# Autodesk Inventor assembly: A Drive
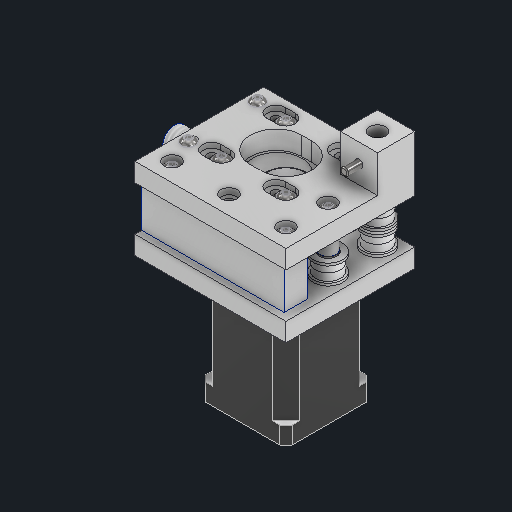
[picture p0: Inventor's stored thumbnail of the model, 512x512]
Saved by Autodesk Inventor 2025.1 (Build 291241020, 241B)
## iProperties
Created: 2025-05-09
Part Number: A Drive
Document SubType Name: Assembly
Designer: AdminForWorker
Title: A Drive
Author: AdminForWorker
## Documents named in this file (9)
- C:\Users\Joshua Eah\Documents\Voron 0.2\CAD\Master Assembly\Motion\AB Drives\A Drive.iam
- C:\Users\Joshua Eah\Documents\Voron 0.2\CAD\Master Assembly\Motion\AB Drives\Motor Assembly.iam
- C:\Users\Joshua Eah\Documents\Voron 0.2\CAD\Machined Parts\AB Drives\A Drive\A Drive Assembly.iam
- C:\Users\Joshua Eah\Documents\Voron 0.2\CAD\Master Assembly\Washers (1).iam
- C:\Users\Joshua Eah\Documents\Voron 0.2\CAD\Master Assembly\Hardware\M3x35 BHCS.ipt
- C:\Users\Joshua Eah\Documents\Voron 0.2\CAD\Master Assembly\Hardware\M3x30 BHCS.ipt
- C:\Users\Joshua Eah\Documents\Voron 0.2\CAD\Master Assembly\Hardware\M3x10 BHCS.ipt
- C:\Users\Joshua Eah\Documents\Voron 0.2\CAD\Master Assembly\Hardware\M3 Hexnut.ipt
- C:\Users\Joshua Eah\Documents\Voron 0.2\CAD\Master Assembly\F623 Stack.iam
## Components (20 placed, 8 different names)
1. Motor Assembly:1 [sub-assembly]
2. A Drive Assembly:1 [sub-assembly]
3. Washers (1):1 [sub-assembly]
4. M3x35 BHCS:1
5. M3x35 BHCS:2
6. M3x35 BHCS:3
7. M3x35 BHCS:4
8. M3x35 BHCS:5
9. M3x35 BHCS:6
10. M3x35 BHCS:7
11. M3x35 BHCS:8
12. M3x30 BHCS:1
13. M3x30 BHCS:2
14. M3x10 BHCS:1
15. M3 Hexnut:1
16. M3 Hexnut:2
17. M3 Hexnut:3
18. F623 Stack:1 [sub-assembly]
19. F623 Stack:2 [sub-assembly]
20. F623 Stack:3 [sub-assembly]
## Relationships (2: Insert 2)
- [Insert]: A Drive Assembly:1 ↔ M3x10 BHCS:1
- [Insert]: A Drive Assembly:1 ↔ M3x35 BHCS:4
